# Autodesk Inventor assembly: motor_replacement
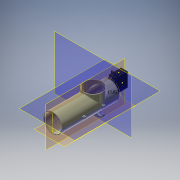
[picture p0: Inventor's stored thumbnail of the model, 180x180]
Saved by Autodesk Inventor 2019 (Build 230136000, 136)
## iProperties
Created: 2019-10-29
Part Number: motor_replacement
Document SubType Name: Assembly
Designer: assman
Author: assman
## Documents named in this file (4)
- D:\Inventor\Projects\CatFeeder\Case\version7\motor_replacement.iam
- D:\Inventor\Projects\CatFeeder\Case\version7\auger_case.ipt
- D:\Inventor\Projects\3party\Servos\MG995.ipt
- D:\Inventor\Projects\CatFeeder\Case\version7\motor_holder.ipt
## Components (3 placed, 3 different names)
1. auger_case:1 — Rigid:1
2. MG995:1 — Rigid:1, Flush:1
3. motor_holder:1 — Flush:1
## Relationships (2: WeldJoint 1, Flush 1)
- Rigid:1 [WeldJoint] (-3.82 mm): auger_case:1 ↔ MG995:1
- Flush:1: MG995:1 ↔ motor_holder:1
